# Autodesk Inventor assembly: Робот
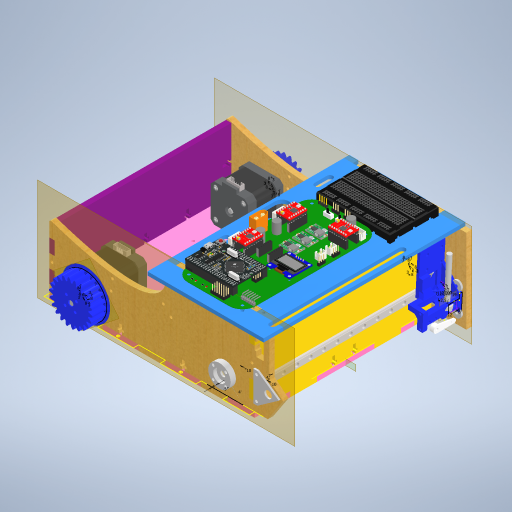
[picture p0: Inventor's stored thumbnail of the model, 512x512]
Saved by Autodesk Inventor 2024.2 (Build 282272000, 272)
## iProperties
Created: 2026-01-27
Part Number: Робот
Document SubType Name: Assembly
Designer: Service
Author: Service
## Documents named in this file (18)
- C:\Users\Service\Documents\Artist-v2\3D\Робот.iam
- C:\Users\Service\Documents\Artist-v2\3D\Низ робота.ipt
- C:\Users\Service\Documents\Artist-v2\3D\бок.ipt
- C:\Users\Service\Documents\Artist-v2\3D\перед.ipt
- C:\Users\Service\Documents\Artist-v2\3D\NEMA17 42-40.ipt
- C:\Users\Service\Documents\Artist-v2\3D\Шестерня.ipt
- C:\Users\Service\Documents\Artist-v2\3D\stl\крепеж валика.ipt
- C:\Users\Service\Documents\Artist-v2\3D\dxf\спиралька.ipt
- C:\Users\Service\Documents\Artist-v2\3D\MGN7.ipt
- C:\Users\Service\Documents\Artist-v2\3D\stl\крышка.ipt
- C:\Users\Service\Documents\Artist-v2\3D\каретка.iam
- C:\Users\Service\Documents\Artist-v2\3D\Проект_ЕТЗ.iam
- C:\Users\Service\Documents\Artist-v2\3D\PROTOBOARD TOP.ipt
- C:\Users\Service\Documents\Artist-v2\3D\stl\задняя стенка.ipt
- C:\Users\Service\Documents\Artist-v2\3D\dxf\крепеж подшипника.ipt
- C:\Users\Service\Documents\Artist-v2\3D\stl\крепеж подшипника.ipt
- C:\Users\Service\Documents\Artist-v2\3D\stl\подшипник не выпадет.ipt
- C:\Users\Service\Documents\Artist-v2\3D\справа бок.ipt
## Components (21 placed, 16 different names)
1. Низ робота:1 — Совмещение:12, Заподлицо:9, Заподлицо:23, Заподлицо:25, Совмещение:47, Заподлицо:26, Заподлицо:27, Совмещение:58
2. перед:1 — Заподлицо:23, Заподлицо:25, Совмещение:51, Заподлицо:30, Совмещение:60, Совмещение:61, Заподлицо:37
3. NEMA17 42-40:1 — Совмещение:4, Совмещение:5, Совмещение:12, Совмещение:14
4. NEMA17 42-40:2 — Совмещение:9
5. Шестерня:1 — Совмещение:13, Совмещение:14
6. Шестерня:2 — Совмещение:42, Совмещение:43
7. Шестерня:3
8. Шестерня:4 — Совмещение:9
9. крепеж валика:1 — Заподлицо:9
10. спиралька:1 — Совмещение:49
11. MGN7:1 — Совмещение:51, Заподлицо:30
12. крышка:1 — Совмещение:55, Совмещение:56, Совмещение:57, Заподлицо:31
13. каретка:1 [sub-assembly] — Совмещение:49
14. Проект_ЕТЗ:1 [sub-assembly] — Совмещение:55, Совмещение:57
15. PROTOBOARD TOP:1 — Совмещение:56
16. задняя стенка:1 — Совмещение:58, Совмещение:59
17. крепеж подшипника:1
18. крепеж подшипника:2 — Заподлицо:33, Заподлицо:34, Заподлицо:36
19. подшипник не выпадет:1 — Заподлицо:35, Заподлицо:36
20. справа бок:1 — Совмещение:60, Совмещение:61, Заподлицо:37
21. бок:1 — Совмещение:4, Совмещение:5, Совмещение:13, Совмещение:42, Совмещение:43, Совмещение:47, Заподлицо:26, Заподлицо:27, Заподлицо:31, Совмещение:59, Заподлицо:33, Заподлицо:34, Заподлицо:35
## Relationships (30: Mate 18, Flush 12)
- Совмещение:4 [Mate]: NEMA17 42-40:1 ↔ бок:1
- Совмещение:5 [Mate]: NEMA17 42-40:1 ↔ бок:1
- Совмещение:9 [Mate]: NEMA17 42-40:2 ↔ Шестерня:4
- Совмещение:12 [Mate]: Низ робота:1 ↔ NEMA17 42-40:1
- Совмещение:13 [Mate]: Шестерня:1 ↔ бок:1
- Совмещение:14 [Mate]: NEMA17 42-40:1 ↔ Шестерня:1
- Заподлицо:9 [Flush]: Низ робота:1 ↔ крепеж валика:1
- Совмещение:42 [Mate]: Шестерня:2 ↔ бок:1
- Совмещение:43 [Mate]: Шестерня:2 ↔ бок:1
- Заподлицо:23 [Flush]: Низ робота:1 ↔ перед:1
- Заподлицо:25 [Flush]: Низ робота:1 ↔ перед:1
- Совмещение:47 [Mate]: Низ робота:1 ↔ бок:1
- Заподлицо:26 [Flush]: Низ робота:1 ↔ бок:1
- Заподлицо:27 [Flush]: Низ робота:1 ↔ бок:1
- Совмещение:49 [Mate]: спиралька:1 ↔ каретка:1
- Совмещение:51 [Mate]: перед:1 ↔ MGN7:1
- Заподлицо:30 [Flush] (64.5 mm): перед:1 ↔ MGN7:1
- Совмещение:55 [Mate] (5 mm): крышка:1 ↔ Проект_ЕТЗ:1
- Совмещение:56 [Mate]: крышка:1 ↔ PROTOBOARD TOP:1
- Совмещение:57 [Mate]: крышка:1 ↔ Проект_ЕТЗ:1
- Заподлицо:31 [Flush]: крышка:1 ↔ бок:1
- Совмещение:58 [Mate]: Низ робота:1 ↔ задняя стенка:1
- Совмещение:59 [Mate]: задняя стенка:1 ↔ бок:1
- Заподлицо:33 [Flush]: крепеж подшипника:2 ↔ бок:1
- Заподлицо:34 [Flush]: крепеж подшипника:2 ↔ бок:1
- Заподлицо:35 [Flush]: подшипник не выпадет:1 ↔ бок:1
- Заподлицо:36 [Flush]: крепеж подшипника:2 ↔ подшипник не выпадет:1
- Совмещение:60 [Mate]: перед:1 ↔ справа бок:1
- Совмещение:61 [Mate]: перед:1 ↔ справа бок:1
- Заподлицо:37 [Flush]: перед:1 ↔ справа бок:1
